# Autodesk Inventor assembly: Assembly1
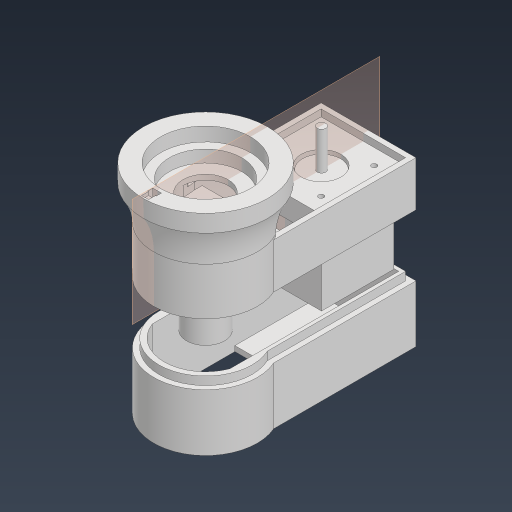
[picture p0: Inventor's stored thumbnail of the model, 512x512]
Saved by Autodesk Inventor 2024 (Build 280153000, 153)
## iProperties
Created: 2025-10-20
Part Number: Assembly1
Document SubType Name: Assembly
Designer: Piter
Author: Piter
## Documents named in this file (5)
- C:\Users\Piter\OneDrive\Pulpit\Robots\david_Arm\Davie-Robot-Arm\3D Models\Base\Assembly1.iam
- C:\Users\Piter\OneDrive\Pulpit\Robots\david_Arm\Davie-Robot-Arm\3D Models\Base\Base_top.ipt
- C:\Users\Piter\OneDrive\Pulpit\Robots\david_Arm\Davie-Robot-Arm\3D Models\Component models\Slip_ring.ipt
- C:\Users\Piter\OneDrive\Pulpit\Robots\david_Arm\Davie-Robot-Arm\3D Models\Base\New_base_v3.ipt
- C:\Users\Piter\OneDrive\Pulpit\Robots\david_Arm\Davie-Robot-Arm\3D Models\Component models\Stepper.ipt
## Components (4 placed, 4 different names)
1. Base_top:1 — Rigid:1, Mate:1, Mate:2, Rigid:2
2. Slip_ring:1 — Rigid:1
3. New_base_v3:1 — Mate:1, Mate:2
4. Stepper:1 — Rigid:2
## Relationships (4: WeldJoint 2, Mate 2)
- Rigid:1 [WeldJoint]: Base_top:1 ↔ Slip_ring:1
- Mate:1: Base_top:1 ↔ New_base_v3:1
- Mate:2: Base_top:1 ↔ New_base_v3:1
- Rigid:2 [WeldJoint]: Base_top:1 ↔ Stepper:1
